# Autodesk Inventor assembly: Plow Part
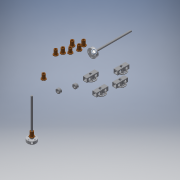
[picture p0: Inventor's stored thumbnail of the model, 180x180]
Saved by Autodesk Inventor 2016 (Build 200138000, 138)
## iProperties
Created: 2015-10-31
Part Number: Plow Part
Document SubType Name: Assembly
Designer: RoboticsUser
Author: RoboticsUser
## Documents named in this file (6)
- C:\Robotics\2015-16 CAD\custom cad parts\Plow Part.iam
- C:\Robotics\2015-16 CAD\COTSParts\Tetrix\Tetrix shaft 100mm.ipt
- C:\Robotics\2015-16 CAD\COTSParts\Tetrix\Bronze bushing.ipt
- C:\Robotics\2015-16 CAD\COTSParts\Tetrix\Tetrix Lego Adapter.ipt
- C:\Robotics\2015-16 CAD\COTSParts\Tetrix\Tetrix shaft collar.ipt
- C:\Robotics\2015-16 CAD\COTSParts\Tetrix\Tetrix Hub - axle_MIR.ipt
## Components (18 placed, 5 different names)
1. Tetrix shaft 100mm:1 — Insert:1, Mate:1
2. Bronze bushing:1
3. Bronze bushing:2
4. Bronze bushing:3
5. Bronze bushing:4
6. Bronze bushing:5
7. Bronze bushing:6
8. Bronze bushing:7 — Mate:1
9. Bronze bushing:8
10. Tetrix shaft 100mm:2 — Insert:2
11. Tetrix Lego Adapter:1
12. Tetrix Lego Adapter:2
13. Tetrix Lego Adapter:3
14. Tetrix Lego Adapter:4
15. Tetrix shaft collar:1
16. Tetrix shaft collar:2
17. Tetrix Hub - axle_MIR:1 — Insert:1
18. Tetrix Hub - axle_MIR:2 — Insert:2
## Relationships (3: Insert 2, Mate 1)
- Insert:1: Tetrix shaft 100mm:1 ↔ Tetrix Hub - axle_MIR:1
- Insert:2: Tetrix shaft 100mm:2 ↔ Tetrix Hub - axle_MIR:2
- Mate:1: Tetrix shaft 100mm:1 ↔ Bronze bushing:7
